# Autodesk Inventor assembly: korob_and_pielers
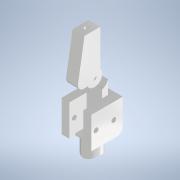
[picture p0: Inventor's stored thumbnail of the model, 180x180]
Saved by Autodesk Inventor 2020 (Build 240168000, 168)
## iProperties
Created: 2020-08-03
Part Number: korob_and_pielers
Document SubType Name: Assembly
Designer: metal
Author: metal
## Documents named in this file (3)
- C:\Polyimide_isolation_cleaner\korob_and_pielers.iam
- C:\Polyimide_isolation_cleaner\korob_3.ipt
- C:\Polyimide_isolation_cleaner\pielers.ipt
## Components (2 placed, 2 different names)
1. korob_3:1 — Rigid:1
2. pielers:1 — Rigid:1
## Relationships (1: WeldJoint 1)
- Rigid:1 [WeldJoint]: korob_3:1 ↔ pielers:1
